# Autodesk Inventor assembly: 000.400 - Первое звено
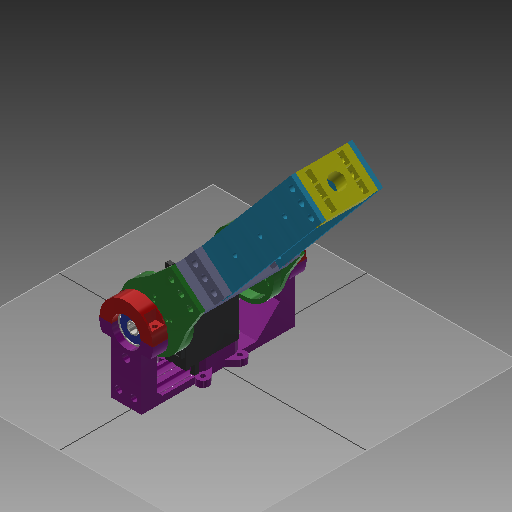
[picture p0: Inventor's stored thumbnail of the model, 512x512]
Saved by Autodesk Inventor 2019 (Build 230136000, 136)
## iProperties
Created: 2020-02-27
Part Number: 000.400 - Первое звено
Material: Типовые
Document SubType Name: Assembly
Designer: Петров Иван
Author: Петров Иван
## Documents named in this file (10)
- E:\IVAN\Ivan_desktop\GitHub\Manipulation_IRS\hardware\5-DOF\000.400 - Первое звено.iam
- E:\IVAN\Ivan_desktop\GitHub\Manipulation_IRS\hardware\5-DOF\000.401 - Держатель 1-ого звена.ipt
- E:\IVAN\Ivan_desktop\GitHub\Manipulation_IRS\hardware\5-DOF\components\tower prone.ipt
- E:\IVAN\Ivan_desktop\GitHub\Manipulation_IRS\hardware\5-DOF\components\Star Horn MG995.ipt
- E:\IVAN\Ivan_desktop\GitHub\Manipulation_IRS\hardware\5-DOF\components\Подшипник 626Z.ipt
- E:\IVAN\Ivan_desktop\GitHub\Manipulation_IRS\hardware\5-DOF\000.402 - Зажим подшипника.ipt
- E:\IVAN\Ivan_desktop\GitHub\Manipulation_IRS\hardware\5-DOF\000.403 - Держатель рычага.ipt
- E:\IVAN\Ivan_desktop\GitHub\Manipulation_IRS\hardware\5-DOF\000.404 - Переходник.ipt
- E:\IVAN\Ivan_desktop\GitHub\Manipulation_IRS\hardware\5-DOF\000.405 - Рычаг.ipt
- E:\IVAN\Ivan_desktop\GitHub\Manipulation_IRS\hardware\5-DOF\000.406 - Проставка.ipt
## Components (13 placed, 9 different names)
1. tower prone:1 — Совмещение:4, Совмещение:5, Совмещение:6, Совмещение:7, Совмещение:8, Совмещение:20
2. Star Horn MG995:1 — Совмещение:4, Совмещение:5, Совмещение:17, Совмещение:19
3. 000.401 - Держатель 1-ого звена:1 — Совмещение:6, Совмещение:7, Совмещение:8, Совмещение:9, Совмещение:11, Заподлицо:12, Совмещение:12, Совмещение:13, Заподлицо:13, Заподлицо:14, Совмещение:14, Совмещение:15, Совмещение:16
4. Подшипник 626Z:1 — Совмещение:9, Заподлицо:12
5. Подшипник 626Z:2 — Совмещение:11, Заподлицо:14, Совмещение:21, Совмещение:22
6. 000.402 - Зажим подшипника:1 — Совмещение:12, Совмещение:13, Заподлицо:13
7. 000.402 - Зажим подшипника:2 — Совмещение:14, Совмещение:15, Совмещение:16
8. 000.403 - Держатель рычага:1 — Совмещение:17, Совмещение:19, Совмещение:20, Совмещение:23, Совмещение:25
9. 000.403 - Держатель рычага:2 — Совмещение:21, Совмещение:22, Совмещение:23, Совмещение:24, Совмещение:26
10. 000.404 - Переходник:1 — Совмещение:24, Совмещение:25, Совмещение:26, Совмещение:27, Совмещение:28, Совмещение:29, Совмещение:30, Совмещение:31, Совмещение:32
11. 000.405 - Рычаг:1 — Совмещение:27, Совмещение:28, Совмещение:29
12. 000.405 - Рычаг:2 — Совмещение:30, Совмещение:31, Совмещение:32, Совмещение:33, Совмещение:34, Совмещение:35
13. 000.406 - Проставка:1 — Совмещение:33, Совмещение:34, Совмещение:35
## Relationships (33: Mate 30, Flush 3)
- Совмещение:4 [Mate]: tower prone:1 ↔ Star Horn MG995:1
- Совмещение:5 [Mate]: tower prone:1 ↔ Star Horn MG995:1
- Совмещение:6 [Mate]: tower prone:1 ↔ 000.401 - Держатель 1-ого звена:1
- Совмещение:7 [Mate]: tower prone:1 ↔ 000.401 - Держатель 1-ого звена:1
- Совмещение:8 [Mate]: tower prone:1 ↔ 000.401 - Держатель 1-ого звена:1
- Совмещение:9 [Mate]: 000.401 - Держатель 1-ого звена:1 ↔ Подшипник 626Z:1
- Совмещение:11 [Mate]: 000.401 - Держатель 1-ого звена:1 ↔ Подшипник 626Z:2
- Заподлицо:12 [Flush]: 000.401 - Держатель 1-ого звена:1 ↔ Подшипник 626Z:1
- Совмещение:12 [Mate]: 000.401 - Держатель 1-ого звена:1 ↔ 000.402 - Зажим подшипника:1
- Совмещение:13 [Mate]: 000.401 - Держатель 1-ого звена:1 ↔ 000.402 - Зажим подшипника:1
- Заподлицо:13 [Flush]: 000.401 - Держатель 1-ого звена:1 ↔ 000.402 - Зажим подшипника:1
- Заподлицо:14 [Flush]: 000.401 - Держатель 1-ого звена:1 ↔ Подшипник 626Z:2
- Совмещение:14 [Mate]: 000.401 - Держатель 1-ого звена:1 ↔ 000.402 - Зажим подшипника:2
- Совмещение:15 [Mate]: 000.401 - Держатель 1-ого звена:1 ↔ 000.402 - Зажим подшипника:2
- Совмещение:16 [Mate]: 000.401 - Держатель 1-ого звена:1 ↔ 000.402 - Зажим подшипника:2
- Совмещение:17 [Mate]: Star Horn MG995:1 ↔ 000.403 - Держатель рычага:1
- Совмещение:19 [Mate]: Star Horn MG995:1 ↔ 000.403 - Держатель рычага:1
- Совмещение:20 [Mate]: tower prone:1 ↔ 000.403 - Держатель рычага:1
- Совмещение:21 [Mate]: Подшипник 626Z:2 ↔ 000.403 - Держатель рычага:2
- Совмещение:22 [Mate]: Подшипник 626Z:2 ↔ 000.403 - Держатель рычага:2
- Совмещение:23 [Mate]: 000.403 - Держатель рычага:1 ↔ 000.403 - Держатель рычага:2
- Совмещение:24 [Mate]: 000.403 - Держатель рычага:2 ↔ 000.404 - Переходник:1
- Совмещение:25 [Mate]: 000.403 - Держатель рычага:1 ↔ 000.404 - Переходник:1
- Совмещение:26 [Mate]: 000.403 - Держатель рычага:2 ↔ 000.404 - Переходник:1
- Совмещение:27 [Mate]: 000.404 - Переходник:1 ↔ 000.405 - Рычаг:1
- Совмещение:28 [Mate]: 000.404 - Переходник:1 ↔ 000.405 - Рычаг:1
- Совмещение:29 [Mate]: 000.404 - Переходник:1 ↔ 000.405 - Рычаг:1
- Совмещение:30 [Mate]: 000.404 - Переходник:1 ↔ 000.405 - Рычаг:2
- Совмещение:31 [Mate]: 000.404 - Переходник:1 ↔ 000.405 - Рычаг:2
- Совмещение:32 [Mate]: 000.404 - Переходник:1 ↔ 000.405 - Рычаг:2
- Совмещение:33 [Mate]: 000.405 - Рычаг:2 ↔ 000.406 - Проставка:1
- Совмещение:34 [Mate]: 000.405 - Рычаг:2 ↔ 000.406 - Проставка:1
- Совмещение:35 [Mate]: 000.405 - Рычаг:2 ↔ 000.406 - Проставка:1
